# Autodesk Inventor assembly: Zespół1
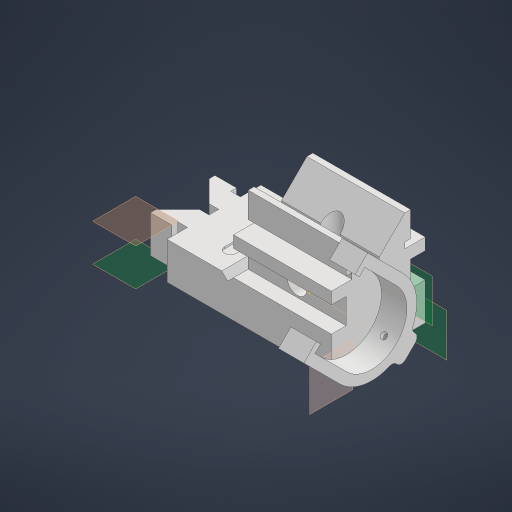
[picture p0: Inventor's stored thumbnail of the model, 512x512]
Saved by Autodesk Inventor 2023 (Build 270158000, 158)
## iProperties
Created: 2023-05-11
Part Number: Zespół1
Document SubType Name: Assembly
Designer: Adam
Author: Adam
## Documents named in this file (3)
- C:\Users\pryst\Desktop\KoNaR\Warsztaty\Mechanika\Projekty\Adam_Prystupa\Zespół1.iam
- C:\Users\pryst\Desktop\KoNaR\Warsztaty\Mechanika\Projekty\Adam_Prystupa\Część30.ipt
- C:\Users\pryst\Desktop\KoNaR\Warsztaty\Mechanika\Projekty\Adam_Prystupa\Część27.ipt
## Components (2 placed, 2 different names)
1. Część30:1 — Kątowe:1, Kątowe:2
2. Część27:1 — Kątowe:1, Kątowe:2
## Relationships (2: Angle 2)
- Kątowe:1 [Angle] (45 deg): Część30:1 ↔ Część27:1
- Kątowe:2 [Angle] (0 deg): Część30:1 ↔ Część27:1
